# Autodesk Inventor assembly: mo0ntaje
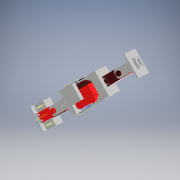
[picture p0: Inventor's stored thumbnail of the model, 180x180]
Saved by Autodesk Inventor 2020 (Build 240168000, 168)
## iProperties
Created: 2020-01-14
Part Number: mo0ntaje
Document SubType Name: Assembly
Designer: Darien
Author: Darien
## Documents named in this file (9)
- D:\Proyectos\Gusano swan\mo0ntaje.iam
- D:\Proyectos\CaMov\Modulo KrYZ mini\motor.ipt
- D:\Proyectos\Gusano swan\soporte.ipt
- D:\Proyectos\Gusano swan\cabeza_s_centro.ipt
- D:\Proyectos\Gusano swan\cabeza_s.ipt
- D:\Proyectos\Gusano swan\base_s.ipt
- D:\Proyectos\Gusano swan\caja_s.ipt
- D:\Proyectos\Gusano swan\tapa_caja.ipt
- D:\Proyectos\Gusano swan\tapa_base.ipt
## Components (15 placed, 8 different names)
1. motor:1 — Mate:3, Flush:3, Flush:4, Mate:13
2. soporte:1 — Mate:3, Flush:3, Flush:4, Rotational:1, Flush:14, Mate:14
3. cabeza_s_centro:1 — Rotational:1, Mate:11, Mate:12, Flush:13
4. motor:2
5. soporte:2
6. cabeza_s:2 — Mate:13, Flush:14, Mate:14, Mate:15, Flush:17, Flush:18
7. base_s:1 — Mate:18, Flush:23, Flush:24, Mate:19, Flush:25, Flush:26
8. motor:3 — Mate:11
9. soporte:3 — Mate:12, Flush:13
10. cabeza_s:1
11. caja_s:2 — Mate:15, Flush:17, Flush:18, Mate:16, Flush:19, Flush:20, Mate:17, Flush:21, Flush:22
12. tapa_caja:1 — Mate:17, Flush:21, Flush:22
13. tapa_caja:2 — Mate:16, Flush:19, Flush:20
14. tapa_base:1 — Mate:18, Flush:23, Flush:24
15. tapa_base:2 — Mate:19, Flush:25, Flush:26
## Relationships (36: Flush 19, Mate 14, RevoluteJoint 3)
- Mate:3: motor:1 ↔ soporte:1
- Flush:3: motor:1 ↔ soporte:1
- Flush:4: motor:1 ↔ soporte:1
- Rotational:1 [RevoluteJoint]: soporte:1 ↔ cabeza_s_centro:1
- [Mate]: motor:2 ↔ soporte:2
- [Flush]: motor:2 ↔ soporte:2
- [Flush]: motor:2 ↔ soporte:2
- [Mate]: motor:2 ↔ base_s:1
- [Mate]: motor:2 ↔ base_s:1
- [Flush]: motor:2 ↔ base_s:1
- [RevoluteJoint]: soporte:2 ↔ cabeza_s:2
- [Mate]: motor:3 ↔ soporte:3
- [Flush]: motor:3 ↔ soporte:3
- [Flush]: motor:3 ↔ soporte:3
- [RevoluteJoint]: soporte:3 ↔ cabeza_s:1
- Mate:11: cabeza_s_centro:1 ↔ motor:3
- Mate:12: cabeza_s_centro:1 ↔ soporte:3
- Flush:13: cabeza_s_centro:1 ↔ soporte:3
- Mate:13: motor:1 ↔ cabeza_s:2
- Flush:14: soporte:1 ↔ cabeza_s:2
- Mate:14: soporte:1 ↔ cabeza_s:2
- Mate:15: cabeza_s:2 ↔ caja_s:2
- Flush:17: cabeza_s:2 ↔ caja_s:2
- Flush:18: cabeza_s:2 ↔ caja_s:2
- Mate:16: caja_s:2 ↔ tapa_caja:2
- Flush:19: caja_s:2 ↔ tapa_caja:2
- Flush:20: caja_s:2 ↔ tapa_caja:2
- Mate:17: caja_s:2 ↔ tapa_caja:1
- Flush:21: caja_s:2 ↔ tapa_caja:1
- Flush:22: caja_s:2 ↔ tapa_caja:1
- Mate:18: base_s:1 ↔ tapa_base:1
- Flush:23: base_s:1 ↔ tapa_base:1
- Flush:24: base_s:1 ↔ tapa_base:1
- Mate:19: base_s:1 ↔ tapa_base:2
- Flush:25: base_s:1 ↔ tapa_base:2
- Flush:26: base_s:1 ↔ tapa_base:2
## Named parameters: d48_d31 = 0 mm, d49_d32 = 0 mm, d50_d36 = 0 mm, d51_d37 = 0 mm, d52_d38 = 0 mm, d53_d39 = 0 mm, d54_d46 = 0 mm, d55_d47 = -177.980059 deg, d59_d31 = 0 mm, d60_d32 = 0 mm, d61_d36 = 0 mm, d65_d46 = 0 mm, d66_d47 = 179.506594 deg
